# Autodesk Inventor assembly: 1310_Drive Coil Assm_V2
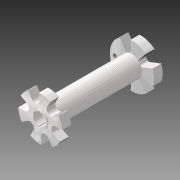
[picture p0: Inventor's stored thumbnail of the model, 180x180]
Saved by Autodesk Inventor 2020 (Build 240168000, 168)
## iProperties
Created: 2019-11-07
Part Number: 1310_Drive Coil Assm_V2
Document SubType Name: Assembly
Designer: RFLab
Author: RFLab
## Documents named in this file (5)
- C:\Users\e22ma\Dropbox\MPI Group Folder\MPS\Inventor_Parts\Parts Numbered - OSMPI\1xxx_Transmit Assembly\13xx_Drive Coil\1310_Drive Coil Assm_V2.iam
- C:\Users\e22ma\Dropbox\MPI Group Folder\MPS\Inventor_Parts\Parts Numbered - OSMPI\1xxx_Transmit Assembly\13xx_Drive Coil\1312A_Drive Coil Second Layer_V1.ipt
- C:\Users\e22ma\Dropbox\MPI Group Folder\MPS\Inventor_Parts\Parts Numbered - OSMPI\1xxx_Transmit Assembly\13xx_Drive Coil\1312B_Drive Coil Second Layer_V1.ipt
- C:\Users\e22ma\Dropbox\MPI Group Folder\MPS\Inventor_Parts\Parts Numbered - OSMPI\1xxx_Transmit Assembly\13xx_Drive Coil\1311_Drive Coil Main Body_V2.ipt
- C:\Users\e22ma\Dropbox\MPI Group Folder\MPS\Inventor_Parts\Parts Numbered - OSMPI\1xxx_Transmit Assembly\13xx_Drive Coil\1313_Drive Coil End_V2.ipt
## Components (4 placed, 4 different names)
1. 1311_Drive Coil Main Body_V2:1 — Mate:2, Mate:3, Mate:5, Mate:6, Mate:9, Mate:10, Mate:11, Mate:13, Flush:1
2. 1312A_Drive Coil Second Layer_V1:1 — Mate:2, Mate:4, Mate:6, Mate:12
3. 1312B_Drive Coil Second Layer_V1:1 — Mate:3, Mate:4, Mate:5
4. 1313_Drive Coil End_V2:1 — Mate:12, Mate:13, Flush:1
## Relationships (11: Mate 10, Flush 1)
- Mate:2: 1311_Drive Coil Main Body_V2:1 ↔ 1312A_Drive Coil Second Layer_V1:1
- Mate:3: 1311_Drive Coil Main Body_V2:1 ↔ 1312B_Drive Coil Second Layer_V1:1
- Mate:4: 1312A_Drive Coil Second Layer_V1:1 ↔ 1312B_Drive Coil Second Layer_V1:1
- Mate:5: 1311_Drive Coil Main Body_V2:1 ↔ 1312B_Drive Coil Second Layer_V1:1
- Mate:6: 1311_Drive Coil Main Body_V2:1 ↔ 1312A_Drive Coil Second Layer_V1:1
- Mate:9: 1311_Drive Coil Main Body_V2:1
- Mate:10: 1311_Drive Coil Main Body_V2:1
- Mate:11: 1311_Drive Coil Main Body_V2:1
- Mate:12: 1312A_Drive Coil Second Layer_V1:1 ↔ 1313_Drive Coil End_V2:1
- Mate:13: 1311_Drive Coil Main Body_V2:1 ↔ 1313_Drive Coil End_V2:1
- Flush:1: 1311_Drive Coil Main Body_V2:1 ↔ 1313_Drive Coil End_V2:1
